# Autodesk Inventor assembly: Peg toy
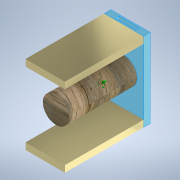
[picture p0: Inventor's stored thumbnail of the model, 180x180]
Saved by Autodesk Inventor 2021 (Build 250183000, 183)
## iProperties
Created: 2020-12-18
Part Number: Peg toy
Document SubType Name: Assembly
Designer: Jawad
Author: Jawad
## Documents named in this file (4)
- E:\OneDrive - UNSW\CAD Files\YOUTUBE tutorial\Peg toy.iam
- E:\OneDrive - UNSW\CAD Files\YOUTUBE tutorial\Peg toy top.ipt
- E:\OneDrive - UNSW\CAD Files\YOUTUBE tutorial\peg toy side.ipt
- E:\OneDrive - UNSW\CAD Files\YOUTUBE tutorial\Peg toy peg.ipt
## Components (4 placed, 3 different names)
1. Peg toy top:1 — Mate:1, Flush:1, Flush:2, Mate:2, Flush:3, Flush:4, Mate:3
2. peg toy side:1 — Mate:2, Flush:3, Flush:4
3. peg toy side:2 — Mate:1, Flush:1, Flush:2
4. Peg toy peg:1 — Mate:3
## Relationships (7: Flush 4, Mate 3)
- Mate:1: Peg toy top:1 ↔ peg toy side:2
- Flush:1: Peg toy top:1 ↔ peg toy side:2
- Flush:2: Peg toy top:1 ↔ peg toy side:2
- Mate:2: Peg toy top:1 ↔ peg toy side:1
- Flush:3: Peg toy top:1 ↔ peg toy side:1
- Flush:4: Peg toy top:1 ↔ peg toy side:1
- Mate:3: Peg toy top:1 ↔ Peg toy peg:1
